# Autodesk Inventor assembly: 000-dribl-v2
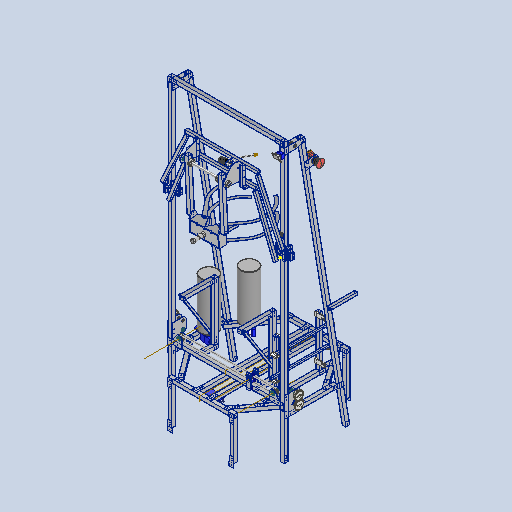
[picture p0: Inventor's stored thumbnail of the model, 512x512]
Saved by Autodesk Inventor 2025.2 (Build 292293000, 293)
## iProperties
Created: 2025-04-03
Part Number: 000-dribl-v2
Document SubType Name: Assembly
Designer: haruy
Author: haruy
## Documents named in this file (56)
- C:\Users\haruy\Documents\ロボコン\NHK2025\cad\nagahisa\dribl\000-dribl-v2.iam
- C:\Users\haruy\Documents\ロボコン\NHK2025\cad\nagahisa\dribl\dribl-v3-Sketch-Base.ipt
- C:\Users\haruy\Documents\ロボコン\NHK2025\cad\nagahisa\dribl\dribl-v1-Plate-5.ipt
- C:\Users\haruy\Documents\ロボコン\NHK2025\cad\nagahisa\dribl\dribl-v1-Plate-3.ipt
- C:\Users\haruy\Documents\ロボコン\NHK2025\cad\nagahisa\dribl\dribl-v1-Plate-4.ipt
- C:\Users\haruy\Documents\ロボコン\NHK2025\cad\nagahisa\dribl\dribl-v3-Plate-1.ipt
- C:\Users\haruy\Documents\ロボコン\NHK2025\cad\nagahisa\dribl\dribl-v3-Plate-2.ipt
- C:\Users\haruy\Documents\ロボコン\NHK2025\cad\nagahisa\dribl\dribl-v3-ASP-arm.ipt
- C:\Users\haruy\Documents\ロボコン\NHK2025\cad\nagahisa\dribl\dribl-v1-Shaft-spesa-57.ipt
- C:\Users\haruy\Documents\ロボコン\NHK2025\cad\nagahisa\dribl\dribl-v1-Plate-8.ipt
- C:\Users\haruy\Documents\ロボコン\NHK2025\cad\000_parts\モーター\robomaster\M2006 P36\RoboMaster M2006 P36\RoboMaster M2006 P36.ipt
- C:\Users\haruy\Documents\ロボコン\NHK2025\cad\nagahisa\dribl\dribl-v3-Plate-6.ipt
- C:\Users\haruy\Documents\ロボコン\NHK2025\cad\nagahisa\dribl\dribl-v3-Plate-7.ipt
- C:\Users\haruy\Documents\ロボコン\NHK2025\cad\nagahisa\dribl\dribl-v3-Plate-8.ipt
- C:\Users\haruy\Documents\ロボコン\NHK2025\cad\nagahisa\dribl\dribl-v3-Plate-9.ipt
- C:\Users\haruy\Documents\ロボコン\NHK2025\cad\nagahisa\dribl\dribl-v3-Plate-10.ipt
- C:\Users\haruy\Documents\ロボコン\NHK2025\cad\nagahisa\dribl\dribl-v3-Plate-11.ipt
- C:\Users\haruy\Documents\ロボコン\NHK2025\cad\nagahisa\dribl\dribl-v3-Plate-12.ipt
- C:\Users\haruy\Documents\ロボコン\NHK2025\cad\nagahisa\dribl\dribl-v3-ASP-1.ipt
- C:\Users\haruy\Documents\ロボコン\NHK2025\cad\nagahisa\dribl\dribl-v1-Plate-14.ipt
- C:\Users\haruy\Documents\ロボコン\NHK2025\cad\nagahisa\dribl\dribl-v1-3DP-P-F.ipt
- C:\Users\haruy\Documents\ロボコン\NHK2025\cad\nagahisa\dribl\roller-Base-v1-petbottle.ipt
- C:\Users\haruy\Documents\ロボコン\NHK2025\cad\nagahisa\dribl\dribl-v3-Plate-13.ipt
- C:\Users\haruy\Documents\ロボコン\NHK2025\cad\nagahisa\dribl\dribl-v3-Plate-14.ipt
- C:\Users\haruy\Documents\ロボコン\NHK2025\cad\nagahisa\base_weel\base_weel-v2-Plate-8.ipt
- C:\Users\haruy\Documents\ロボコン\NHK2025\cad\nagahisa\dribl\dribl-v3-ASP-2.ipt
- C:\Users\haruy\Documents\ロボコン\NHK2025\cad\nagahisa\base_weel\base_weel-v2-POM-pc-F-1.ipt
- C:\Users\haruy\Documents\ロボコン\NHK2025\cad\nagahisa\base_weel\base_weel-v2-POM-pc-F-2.ipt
- C:\Users\haruy\Documents\ロボコン\NHK2025\cad\nagahisa\dribl\dribl-v3-Plate-15.ipt
- C:\Users\haruy\Documents\ロボコン\NHK2025\cad\nagahisa\dribl\dribl-v1-Plate-13.ipt
- C:\Users\haruy\Documents\ロボコン\NHK2025\cad\000_parts\回路関連\EMO\emo_sa.ipt
- C:\Users\haruy\Documents\ロボコン\NHK2025\cad\nagahisa\dribl\dribl-v3-3DP-1.ipt
- C:\Users\haruy\Documents\ロボコン\NHK2025\cad\nagahisa\dribl\dribl-v3-Plate-16.ipt
- C:\Users\haruy\Documents\ロボコン\NHK2025\cad\nagahisa\dribl\000-dribl-v2\デザイン アクセラレータ\歯付きベルト伝達1.iam
- C:\Users\haruy\Documents\ロボコン\NHK2025\cad\000_parts\ベアリング\10\bear_10_15_sn.ipt
- C:\Users\haruy\Documents\ロボコン\NHK2025\cad\nagahisa\belt_liner\SCBRJ10-13.iam
- C:\Users\haruy\Documents\ロボコン\NHK2025\cad\nagahisa\dribl\dribl-v1-Plate-12.ipt
- C:\Users\haruy\Documents\ロボコン\NHK2025\cad\nagahisa\dribl\dribl-v1-3DP-l-F-1.ipt
- C:\Users\haruy\Documents\ロボコン\NHK2025\cad\000_parts\センサー\VX-012-1A3\VX-012-1A3\VX-012-1A3.iam
- C:\Users\haruy\Documents\ロボコン\NHK2025\cad\nagahisa\dribl\R2-Rzvector\TH22_bearing_12_18_19.5_sn.ipt
- C:\Users\haruy\Documents\ロボコン\NHK2025\cad\nagahisa\dribl\SCSNAJ12-16b.ipt
- C:\Users\haruy\Documents\ロボコン\NHK2025\cad\nagahisa\dribl\dribl-v1-Shaft-2.ipt
- C:\Users\haruy\Documents\ロボコン\NHK2025\cad\nagahisa\dribl\dribl-v3-3DP-2.ipt
- C:\Users\haruy\Documents\ロボコン\NHK2025\cad\000_parts\センサー\realsense\D435i_Solid.ipt
- C:\Users\haruy\Documents\ロボコン\NHK2025\cad\nagahisa\dribl\R2-Rzvector\bear_f8_12_sa.ipt
- C:\Users\haruy\Documents\ロボコン\NHK2025\cad\nagahisa\dribl\R2-Rzvector\bear_10_15_sn.ipt
- C:\Users\haruy\Documents\ロボコン\NHK2025\cad\nagahisa\dribl\SCTW12.iam
- C:\Users\haruy\Documents\ロボコン\NHK2025\cad\nagahisa\base_weel\SCSWA8-8.iam
- C:\Users\haruy\Documents\ロボコン\NHK2025\cad\nagahisa\belt_liner\SSCSW10-10b.ipt
- C:\Users\haruy\Documents\ロボコン\NHK2025\cad\nagahisa\dribl\000-dribl-v2\デザイン アクセラレータ\平歯車1.iam
- C:\Users\haruy\Documents\ロボコン\NHK2025\cad\nagahisa\dribl\000-dribl-v2\デザイン アクセラレータ\平歯車2.iam
- C:\Users\haruy\Documents\ロボコン\NHK2025\cad\nagahisa\hand\grab\hand-grab-v5-Plate-6.ipt
- C:\Users\haruy\Documents\ロボコン\NHK2025\cad\nagahisa\hand\grab\hand-grab-v5-Plate-7.ipt
- C:\Users\haruy\Documents\ロボコン\NHK2025\cad\nagahisa\hand\grab\000-hand-grab-v5.iam
- C:\Users\haruy\Documents\ロボコン\NHK2025\cad\nagahisa\hand\grab\hand-grab-v5-ASP-1.ipt
- C:\Users\haruy\Documents\ロボコン\NHK2025\cad\nagahisa\dribl\SCSW12-10.iam
## Components (113 placed, 53 different names)
1. dribl-v3-Sketch-Base:1 — 挿入:10, 挿入:11, 挿入:12, 挿入:13, 挿入:14, 挿入:15, 挿入:16, 挿入:17, 挿入:18, 挿入:19, 挿入:20, 挿入:21, 挿入:22, 挿入:23, 挿入:24, 挿入:25, 挿入:26, 挿入:27, 挿入:28, 挿入:29, 挿入:30, 挿入:31, 挿入:32, 挿入:33, 正接:1, 正接:2, 正接:3, 正接:4, 挿入:44, 挿入:45, 挿入:46, 挿入:47, 挿入:48, 挿入:49, 挿入:50, 挿入:51, 挿入:52, 挿入:53, 挿入:56, 挿入:57, 挿入:58, 挿入:59, 挿入:60, 挿入:61, 挿入:62, 挿入:63, 挿入:64, 挿入:65, 挿入:70, 挿入:71, 挿入:72, 挿入:73, 挿入:74, 挿入:75, 挿入:76, 挿入:77, 挿入:78, 挿入:79, 挿入:80, 挿入:81, 挿入:82, 挿入:83, 挿入:84, 挿入:85, 挿入:86, 挿入:87, 挿入:88, 挿入:89, 挿入:90, 挿入:91, 挿入:92, 挿入:93, 挿入:94, 挿入:95, 挿入:96, 挿入:97, メイト:3, メイト:4, メイト:5, メイト:6, 挿入:102, 挿入:103, 挿入:104, 挿入:105, 挿入:106, 挿入:107, 挿入:108, 挿入:109, 挿入:128, 挿入:129, 挿入:130, 挿入:131, 挿入:132, 挿入:133, 挿入:134, 挿入:135, 挿入:137, 挿入:138, 挿入:139, 挿入:140, フラッシュ:1, 挿入:149, 挿入:150, 挿入:151, 挿入:152, 挿入:163, 挿入:164
2. dribl-v1-Plate-5:1 — 挿入:12, 挿入:13, 挿入:173, 挿入:175
3. dribl-v1-Plate-5:2 — 挿入:10, 挿入:11, 挿入:174, 挿入:176
4. dribl-v1-Plate-3:1 — 挿入:14, 挿入:15, 挿入:167, 挿入:183
5. dribl-v1-Plate-4:1 — 挿入:16, 挿入:17, 挿入:168
6. dribl-v3-Plate-1:1 — 挿入:18, 挿入:19, 挿入:172
7. dribl-v3-Plate-1:2 — 挿入:20, 挿入:21, 挿入:171
8. dribl-v3-Plate-1:3 — 挿入:22, 挿入:23, 挿入:170
9. dribl-v3-Plate-1:4 — 挿入:24, 挿入:25, 挿入:169
10. dribl-v3-Plate-2:1 — 挿入:26, 挿入:27, 挿入:179
11. dribl-v3-Plate-2:2 — 挿入:28, 挿入:29, 挿入:180
12. dribl-v3-Plate-2:3 — 挿入:32, 挿入:33, 挿入:177
13. dribl-v3-Plate-2:4 — 挿入:30, 挿入:31, 挿入:178
14. dribl-v3-ASP-arm:1 — 正接:1, 正接:2, 正接:3, 正接:4, 挿入:202, 挿入:203, 挿入:204, 挿入:205
15. dribl-v1-Shaft-spesa-57:1 — 挿入:41, 挿入:206
16. dribl-v1-Shaft-spesa-57:2 — 挿入:208
17. dribl-v1-Shaft-spesa-57:3 — 挿入:42, 挿入:207
18. dribl-v1-Plate-8:1 — 挿入:41, 挿入:42, 挿入:43, 挿入:208
19. RoboMaster M2006 P36:1 — 挿入:43
20. dribl-v3-Plate-6:1 — 挿入:44, 挿入:45
21. dribl-v3-Plate-6:2 — 挿入:50, 挿入:51
22. dribl-v3-Plate-6:3 — 挿入:48, 挿入:49
23. dribl-v3-Plate-6:4 — 挿入:46, 挿入:47
24. dribl-v3-Plate-7:1 — 挿入:52, 挿入:53
25. dribl-v3-Plate-7:4 — 挿入:56, 挿入:57
26. dribl-v3-Plate-8:1 — 挿入:58, 挿入:59
27. dribl-v3-Plate-8:2 — 挿入:60, 挿入:61
28. dribl-v3-Plate-9:1 — 挿入:62, 挿入:63
29. dribl-v3-Plate-9:3 — 挿入:64, 挿入:65
30. dribl-v3-Plate-10:1 — 挿入:72, 挿入:73
31. dribl-v3-Plate-10:2 — 挿入:74, 挿入:75
32. dribl-v3-Plate-10:3 — 挿入:70, 挿入:71
33. dribl-v3-Plate-10:4 — 挿入:76, 挿入:77
34. dribl-v3-Plate-11:1 — 挿入:78, 挿入:79
35. dribl-v3-Plate-11:2 — 挿入:82, 挿入:83
36. dribl-v3-Plate-11:3 — 挿入:80, 挿入:81
37. dribl-v3-Plate-11:4 — 挿入:84, 挿入:85
38. dribl-v3-Plate-11:5 — 挿入:88, 挿入:89
39. dribl-v3-Plate-11:6 — 挿入:86, 挿入:87
40. dribl-v3-Plate-12:1 — 挿入:90, 挿入:91
41. dribl-v3-Plate-12:2 — 挿入:92, 挿入:93
42. dribl-v3-ASP-1:1 — 挿入:98, 挿入:99
43. dribl-v1-Plate-14:1 — 挿入:96, 挿入:97
44. dribl-v1-Plate-14:2 — 挿入:94, 挿入:95, 挿入:98, 挿入:99
45. dribl-v1-3DP-P-F:1 — 挿入:100, メイト:5, メイト:6
46. roller-Base-v1-petbottle:1 — 挿入:100
47. dribl-v1-3DP-P-F:2 — メイト:3, メイト:4, 挿入:101
48. roller-Base-v1-petbottle:2 — 挿入:101
49. dribl-v3-Plate-13:1 — 挿入:102, 挿入:103
50. dribl-v3-Plate-14:1 — 挿入:104, 挿入:105
51. base_weel-v2-Plate-8:1 — 挿入:106, 挿入:107, 挿入:110, 挿入:111
52. base_weel-v2-Plate-8:2 — 挿入:108, 挿入:109
53. dribl-v3-ASP-2:1 — 挿入:110, 挿入:111, 挿入:112, 挿入:113, 挿入:114, 挿入:115, 挿入:116, 挿入:117, 挿入:118, 挿入:119, 挿入:120, 挿入:121, 挿入:122, 挿入:123, 挿入:124, 挿入:125, 挿入:126, 挿入:127
54. base_weel-v2-POM-pc-F-1:1 — 挿入:112, 挿入:113
55. base_weel-v2-POM-pc-F-1:2 — 挿入:114, 挿入:115
56. base_weel-v2-POM-pc-F-2:1 — 挿入:118, 挿入:119
57. base_weel-v2-POM-pc-F-2:2 — 挿入:116, 挿入:117
58. base_weel-v2-POM-pc-F-2:3 — 挿入:122, 挿入:123
59. base_weel-v2-POM-pc-F-2:4 — 挿入:120, 挿入:121
60. base_weel-v2-POM-pc-F-1:3 — 挿入:126, 挿入:127
61. base_weel-v2-POM-pc-F-1:4 — 挿入:124, 挿入:125
62. dribl-v3-Plate-15:1 — 挿入:128, 挿入:129
63. dribl-v3-Plate-15:2 — 挿入:130, 挿入:131
64. dribl-v3-Plate-11:7 — 挿入:132, 挿入:133
65. dribl-v1-Plate-13:1 — 挿入:134, 挿入:135, 挿入:136
66. emo_sa:1 — 挿入:136
67. dribl-v3-3DP-1:1 — 挿入:139, 挿入:140, 挿入:143, 挿入:144
68. dribl-v3-3DP-1:2 — 挿入:137, 挿入:138, 挿入:141, 挿入:142
69. dribl-v3-Plate-16:1 — 挿入:143, 挿入:144
70. dribl-v3-Plate-16:2 — 挿入:141, 挿入:142
71. 歯付きベルト伝達:1 [sub-assembly] — 挿入:145, 挿入:146
72. bear_10_15_sn:1 — 挿入:145, 挿入:147
73. bear_10_15_sn:2 — 挿入:146, 挿入:148
74. SCBRJ10-13:1 [sub-assembly] — 挿入:147
75. SCBRJ10-13:2 [sub-assembly] — 挿入:148
76. dribl-v1-Plate-12:1 — 挿入:149, 挿入:150, 挿入:155, 挿入:156
77. dribl-v1-3DP-l-F-1:1 — 挿入:151, 挿入:152, 挿入:153, 挿入:154
78. VX-012-1A3:1 [sub-assembly] — 挿入:153, 挿入:154
79. VX-012-1A3:2 [sub-assembly] — 挿入:155, 挿入:156
80. TH22_bearing_12_18_19.5_sn:1 — 挿入:160, 挿入:210
81. TH22_bearing_12_18_19.5_sn:2 — 挿入:194, 挿入:209
82. SCSNAJ12-16b:1 — 挿入:194
83. SCSNAJ12-16b:2 — 挿入:160, 挿入:195
84. dribl-v1-Shaft-2:1 — 挿入:195
85. dribl-v3-3DP-2:1 — 挿入:163, 挿入:164, 挿入:165, 挿入:166
86. D435i_Solid:1 — 挿入:165, 挿入:166
87. TH22_bearing_12_18_19.5_sn:3 — 挿入:167, 挿入:184
88. TH22_bearing_12_18_19.5_sn:4 — 挿入:168
89. TH22_bearing_12_18_19.5_sn:5 — 挿入:170
90. TH22_bearing_12_18_19.5_sn:6 — 挿入:169
91. TH22_bearing_12_18_19.5_sn:7 — 挿入:171
92. TH22_bearing_12_18_19.5_sn:8 — 挿入:172
93. TH22_bearing_12_18_19.5_sn:9 — 挿入:173
94. TH22_bearing_12_18_19.5_sn:10 — 挿入:174, 挿入:181
95. bear_f8_12_sa:1 — 挿入:175
96. bear_f8_12_sa:2 — 挿入:176, 挿入:182
97. bear_10_15_sn:3 — 挿入:178
98. bear_10_15_sn:4 — 挿入:177
99. bear_10_15_sn:5 — 挿入:179
100. bear_10_15_sn:6 — 挿入:180
101. SCTW12:1 [sub-assembly] — 挿入:181, メイト:12
102. SCSWA8-8:1 [sub-assembly] — 挿入:182, メイト:10, メイト:11
103. SSCSW10-10b:1 — 挿入:183, メイト:9
104. SCTW12:2 [sub-assembly] — 挿入:184, メイト:7, メイト:8
105. 平歯車:1 [sub-assembly] — メイト:7, メイト:8, メイト:9
106. 平歯車:2 [sub-assembly] — メイト:10, メイト:11, メイト:12
107. hand-grab-v5-Plate-6:1 — 挿入:202, 挿入:203, 挿入:206, 挿入:207, 挿入:210, 挿入:211
108. hand-grab-v5-Plate-7:1 — 挿入:204, 挿入:205, 挿入:209
109. 000-hand-grab-v5:1 [sub-assembly] — 挿入:196, 挿入:197, 挿入:198, 挿入:199
110. hand-grab-v5-ASP-1:1 — 挿入:196, 挿入:197, 挿入:200
111. hand-grab-v5-ASP-1:2 — 挿入:198, 挿入:199, 挿入:201, 挿入:211
112. SCSW12-10:1 [sub-assembly] — 挿入:201
113. SCSW12-10:2 [sub-assembly] — 挿入:200
## Relationships (190: Insert 175, Mate 10, Tangent 4, Flush 1)
- 挿入:10 [Insert]: dribl-v3-Sketch-Base:1 ↔ dribl-v1-Plate-5:2
- 挿入:11 [Insert]: dribl-v3-Sketch-Base:1 ↔ dribl-v1-Plate-5:2
- 挿入:12 [Insert]: dribl-v3-Sketch-Base:1 ↔ dribl-v1-Plate-5:1
- 挿入:13 [Insert]: dribl-v3-Sketch-Base:1 ↔ dribl-v1-Plate-5:1
- 挿入:14 [Insert]: dribl-v3-Sketch-Base:1 ↔ dribl-v1-Plate-3:1
- 挿入:15 [Insert]: dribl-v3-Sketch-Base:1 ↔ dribl-v1-Plate-3:1
- 挿入:16 [Insert]: dribl-v3-Sketch-Base:1 ↔ dribl-v1-Plate-4:1
- 挿入:17 [Insert]: dribl-v3-Sketch-Base:1 ↔ dribl-v1-Plate-4:1
- 挿入:18 [Insert]: dribl-v3-Sketch-Base:1 ↔ dribl-v3-Plate-1:1
- 挿入:19 [Insert]: dribl-v3-Sketch-Base:1 ↔ dribl-v3-Plate-1:1
- 挿入:20 [Insert]: dribl-v3-Sketch-Base:1 ↔ dribl-v3-Plate-1:2
- 挿入:21 [Insert]: dribl-v3-Sketch-Base:1 ↔ dribl-v3-Plate-1:2
- 挿入:22 [Insert]: dribl-v3-Sketch-Base:1 ↔ dribl-v3-Plate-1:3
- 挿入:23 [Insert]: dribl-v3-Sketch-Base:1 ↔ dribl-v3-Plate-1:3
- 挿入:24 [Insert]: dribl-v3-Sketch-Base:1 ↔ dribl-v3-Plate-1:4
- 挿入:25 [Insert]: dribl-v3-Sketch-Base:1 ↔ dribl-v3-Plate-1:4
- 挿入:26 [Insert]: dribl-v3-Sketch-Base:1 ↔ dribl-v3-Plate-2:1
- 挿入:27 [Insert]: dribl-v3-Sketch-Base:1 ↔ dribl-v3-Plate-2:1
- 挿入:28 [Insert]: dribl-v3-Sketch-Base:1 ↔ dribl-v3-Plate-2:2
- 挿入:29 [Insert]: dribl-v3-Sketch-Base:1 ↔ dribl-v3-Plate-2:2
- 挿入:30 [Insert]: dribl-v3-Sketch-Base:1 ↔ dribl-v3-Plate-2:4
- 挿入:31 [Insert]: dribl-v3-Sketch-Base:1 ↔ dribl-v3-Plate-2:4
- 挿入:32 [Insert]: dribl-v3-Sketch-Base:1 ↔ dribl-v3-Plate-2:3
- 挿入:33 [Insert]: dribl-v3-Sketch-Base:1 ↔ dribl-v3-Plate-2:3
- 正接:1 [Tangent]: dribl-v3-Sketch-Base:1 ↔ dribl-v3-ASP-arm:1
- 正接:2 [Tangent]: dribl-v3-Sketch-Base:1 ↔ dribl-v3-ASP-arm:1
- 正接:3 [Tangent]: dribl-v3-Sketch-Base:1 ↔ dribl-v3-ASP-arm:1
- 正接:4 [Tangent]: dribl-v3-Sketch-Base:1 ↔ dribl-v3-ASP-arm:1
- 挿入:41 [Insert]: dribl-v1-Shaft-spesa-57:1 ↔ dribl-v1-Plate-8:1
- 挿入:42 [Insert]: dribl-v1-Shaft-spesa-57:3 ↔ dribl-v1-Plate-8:1
- 挿入:43 [Insert]: dribl-v1-Plate-8:1 ↔ RoboMaster M2006 P36:1
- 挿入:44 [Insert]: dribl-v3-Sketch-Base:1 ↔ dribl-v3-Plate-6:1
- 挿入:45 [Insert]: dribl-v3-Sketch-Base:1 ↔ dribl-v3-Plate-6:1
- 挿入:46 [Insert]: dribl-v3-Sketch-Base:1 ↔ dribl-v3-Plate-6:4
- 挿入:47 [Insert]: dribl-v3-Sketch-Base:1 ↔ dribl-v3-Plate-6:4
- 挿入:48 [Insert]: dribl-v3-Sketch-Base:1 ↔ dribl-v3-Plate-6:3
- 挿入:49 [Insert]: dribl-v3-Sketch-Base:1 ↔ dribl-v3-Plate-6:3
- 挿入:50 [Insert]: dribl-v3-Sketch-Base:1 ↔ dribl-v3-Plate-6:2
- 挿入:51 [Insert]: dribl-v3-Sketch-Base:1 ↔ dribl-v3-Plate-6:2
- 挿入:52 [Insert]: dribl-v3-Sketch-Base:1 ↔ dribl-v3-Plate-7:1
- 挿入:53 [Insert]: dribl-v3-Sketch-Base:1 ↔ dribl-v3-Plate-7:1
- 挿入:56 [Insert]: dribl-v3-Sketch-Base:1 ↔ dribl-v3-Plate-7:4
- 挿入:57 [Insert]: dribl-v3-Sketch-Base:1 ↔ dribl-v3-Plate-7:4
- 挿入:58 [Insert]: dribl-v3-Sketch-Base:1 ↔ dribl-v3-Plate-8:1
- 挿入:59 [Insert]: dribl-v3-Sketch-Base:1 ↔ dribl-v3-Plate-8:1
- 挿入:60 [Insert]: dribl-v3-Sketch-Base:1 ↔ dribl-v3-Plate-8:2
- 挿入:61 [Insert]: dribl-v3-Sketch-Base:1 ↔ dribl-v3-Plate-8:2
- 挿入:62 [Insert]: dribl-v3-Sketch-Base:1 ↔ dribl-v3-Plate-9:1
- 挿入:63 [Insert]: dribl-v3-Sketch-Base:1 ↔ dribl-v3-Plate-9:1
- 挿入:64 [Insert]: dribl-v3-Sketch-Base:1 ↔ dribl-v3-Plate-9:3
- 挿入:65 [Insert]: dribl-v3-Sketch-Base:1 ↔ dribl-v3-Plate-9:3
- 挿入:70 [Insert]: dribl-v3-Sketch-Base:1 ↔ dribl-v3-Plate-10:3
- 挿入:71 [Insert]: dribl-v3-Sketch-Base:1 ↔ dribl-v3-Plate-10:3
- 挿入:72 [Insert]: dribl-v3-Sketch-Base:1 ↔ dribl-v3-Plate-10:1
- 挿入:73 [Insert]: dribl-v3-Sketch-Base:1 ↔ dribl-v3-Plate-10:1
- 挿入:74 [Insert]: dribl-v3-Sketch-Base:1 ↔ dribl-v3-Plate-10:2
- 挿入:75 [Insert]: dribl-v3-Sketch-Base:1 ↔ dribl-v3-Plate-10:2
- 挿入:76 [Insert]: dribl-v3-Sketch-Base:1 ↔ dribl-v3-Plate-10:4
- 挿入:77 [Insert]: dribl-v3-Sketch-Base:1 ↔ dribl-v3-Plate-10:4
- 挿入:78 [Insert]: dribl-v3-Sketch-Base:1 ↔ dribl-v3-Plate-11:1
- 挿入:79 [Insert]: dribl-v3-Sketch-Base:1 ↔ dribl-v3-Plate-11:1
- 挿入:80 [Insert]: dribl-v3-Sketch-Base:1 ↔ dribl-v3-Plate-11:3
- 挿入:81 [Insert]: dribl-v3-Sketch-Base:1 ↔ dribl-v3-Plate-11:3
- 挿入:82 [Insert]: dribl-v3-Sketch-Base:1 ↔ dribl-v3-Plate-11:2
- 挿入:83 [Insert]: dribl-v3-Sketch-Base:1 ↔ dribl-v3-Plate-11:2
- 挿入:84 [Insert]: dribl-v3-Sketch-Base:1 ↔ dribl-v3-Plate-11:4
- 挿入:85 [Insert]: dribl-v3-Sketch-Base:1 ↔ dribl-v3-Plate-11:4
- 挿入:86 [Insert]: dribl-v3-Sketch-Base:1 ↔ dribl-v3-Plate-11:6
- 挿入:87 [Insert]: dribl-v3-Sketch-Base:1 ↔ dribl-v3-Plate-11:6
- 挿入:88 [Insert]: dribl-v3-Sketch-Base:1 ↔ dribl-v3-Plate-11:5
- 挿入:89 [Insert]: dribl-v3-Sketch-Base:1 ↔ dribl-v3-Plate-11:5
- 挿入:90 [Insert]: dribl-v3-Sketch-Base:1 ↔ dribl-v3-Plate-12:1
- 挿入:91 [Insert]: dribl-v3-Sketch-Base:1 ↔ dribl-v3-Plate-12:1
- 挿入:92 [Insert]: dribl-v3-Sketch-Base:1 ↔ dribl-v3-Plate-12:2
- 挿入:93 [Insert]: dribl-v3-Sketch-Base:1 ↔ dribl-v3-Plate-12:2
- 挿入:94 [Insert]: dribl-v3-Sketch-Base:1 ↔ dribl-v1-Plate-14:2
- 挿入:95 [Insert]: dribl-v3-Sketch-Base:1 ↔ dribl-v1-Plate-14:2
- 挿入:96 [Insert]: dribl-v3-Sketch-Base:1 ↔ dribl-v1-Plate-14:1
- 挿入:97 [Insert]: dribl-v3-Sketch-Base:1 ↔ dribl-v1-Plate-14:1
- 挿入:98 [Insert]: dribl-v3-ASP-1:1 ↔ dribl-v1-Plate-14:2
- 挿入:99 [Insert]: dribl-v3-ASP-1:1 ↔ dribl-v1-Plate-14:2
- 挿入:100 [Insert]: dribl-v1-3DP-P-F:1 ↔ roller-Base-v1-petbottle:1
- メイト:3 [Mate]: dribl-v3-Sketch-Base:1 ↔ dribl-v1-3DP-P-F:2
- メイト:4 [Mate]: dribl-v3-Sketch-Base:1 ↔ dribl-v1-3DP-P-F:2
- 挿入:101 [Insert]: dribl-v1-3DP-P-F:2 ↔ roller-Base-v1-petbottle:2
- メイト:5 [Mate]: dribl-v3-Sketch-Base:1 ↔ dribl-v1-3DP-P-F:1
- メイト:6 [Mate]: dribl-v3-Sketch-Base:1 ↔ dribl-v1-3DP-P-F:1
- 挿入:102 [Insert]: dribl-v3-Sketch-Base:1 ↔ dribl-v3-Plate-13:1
- 挿入:103 [Insert]: dribl-v3-Sketch-Base:1 ↔ dribl-v3-Plate-13:1
- 挿入:104 [Insert]: dribl-v3-Sketch-Base:1 ↔ dribl-v3-Plate-14:1
- 挿入:105 [Insert]: dribl-v3-Sketch-Base:1 ↔ dribl-v3-Plate-14:1
- 挿入:106 [Insert]: dribl-v3-Sketch-Base:1 ↔ base_weel-v2-Plate-8:1
- 挿入:107 [Insert]: dribl-v3-Sketch-Base:1 ↔ base_weel-v2-Plate-8:1
- 挿入:108 [Insert]: dribl-v3-Sketch-Base:1 ↔ base_weel-v2-Plate-8:2
- 挿入:109 [Insert]: dribl-v3-Sketch-Base:1 ↔ base_weel-v2-Plate-8:2
- 挿入:110 [Insert]: base_weel-v2-Plate-8:1 ↔ dribl-v3-ASP-2:1
- 挿入:111 [Insert]: base_weel-v2-Plate-8:1 ↔ dribl-v3-ASP-2:1
- 挿入:112 [Insert]: dribl-v3-ASP-2:1 ↔ base_weel-v2-POM-pc-F-1:1
- 挿入:113 [Insert]: dribl-v3-ASP-2:1 ↔ base_weel-v2-POM-pc-F-1:1
- 挿入:114 [Insert]: dribl-v3-ASP-2:1 ↔ base_weel-v2-POM-pc-F-1:2
- 挿入:115 [Insert]: dribl-v3-ASP-2:1 ↔ base_weel-v2-POM-pc-F-1:2
- 挿入:116 [Insert]: dribl-v3-ASP-2:1 ↔ base_weel-v2-POM-pc-F-2:2
- 挿入:117 [Insert]: dribl-v3-ASP-2:1 ↔ base_weel-v2-POM-pc-F-2:2
- 挿入:118 [Insert]: dribl-v3-ASP-2:1 ↔ base_weel-v2-POM-pc-F-2:1
- 挿入:119 [Insert]: dribl-v3-ASP-2:1 ↔ base_weel-v2-POM-pc-F-2:1
- 挿入:120 [Insert]: dribl-v3-ASP-2:1 ↔ base_weel-v2-POM-pc-F-2:4
- 挿入:121 [Insert]: dribl-v3-ASP-2:1 ↔ base_weel-v2-POM-pc-F-2:4
- 挿入:122 [Insert]: dribl-v3-ASP-2:1 ↔ base_weel-v2-POM-pc-F-2:3
- 挿入:123 [Insert]: dribl-v3-ASP-2:1 ↔ base_weel-v2-POM-pc-F-2:3
- 挿入:124 [Insert]: dribl-v3-ASP-2:1 ↔ base_weel-v2-POM-pc-F-1:4
- 挿入:125 [Insert]: dribl-v3-ASP-2:1 ↔ base_weel-v2-POM-pc-F-1:4
- 挿入:126 [Insert]: dribl-v3-ASP-2:1 ↔ base_weel-v2-POM-pc-F-1:3
- 挿入:127 [Insert]: dribl-v3-ASP-2:1 ↔ base_weel-v2-POM-pc-F-1:3
- 挿入:128 [Insert]: dribl-v3-Sketch-Base:1 ↔ dribl-v3-Plate-15:1
- 挿入:129 [Insert]: dribl-v3-Sketch-Base:1 ↔ dribl-v3-Plate-15:1
- 挿入:130 [Insert]: dribl-v3-Sketch-Base:1 ↔ dribl-v3-Plate-15:2
- 挿入:131 [Insert]: dribl-v3-Sketch-Base:1 ↔ dribl-v3-Plate-15:2
- 挿入:132 [Insert]: dribl-v3-Sketch-Base:1 ↔ dribl-v3-Plate-11:7
- 挿入:133 [Insert]: dribl-v3-Sketch-Base:1 ↔ dribl-v3-Plate-11:7
- 挿入:134 [Insert]: dribl-v3-Sketch-Base:1 ↔ dribl-v1-Plate-13:1
- 挿入:135 [Insert]: dribl-v3-Sketch-Base:1 ↔ dribl-v1-Plate-13:1
- 挿入:136 [Insert]: dribl-v1-Plate-13:1 ↔ emo_sa:1
- 挿入:137 [Insert]: dribl-v3-Sketch-Base:1 ↔ dribl-v3-3DP-1:2
- 挿入:138 [Insert]: dribl-v3-Sketch-Base:1 ↔ dribl-v3-3DP-1:2
- 挿入:139 [Insert]: dribl-v3-Sketch-Base:1 ↔ dribl-v3-3DP-1:1
- 挿入:140 [Insert]: dribl-v3-Sketch-Base:1 ↔ dribl-v3-3DP-1:1
- 挿入:141 [Insert]: dribl-v3-3DP-1:2 ↔ dribl-v3-Plate-16:2
- 挿入:142 [Insert]: dribl-v3-3DP-1:2 ↔ dribl-v3-Plate-16:2
- 挿入:143 [Insert]: dribl-v3-3DP-1:1 ↔ dribl-v3-Plate-16:1
- 挿入:144 [Insert]: dribl-v3-3DP-1:1 ↔ dribl-v3-Plate-16:1
- フラッシュ:1 [Flush] (-10 mm): dribl-v3-Sketch-Base:1
- 挿入:145 [Insert]: 歯付きベルト伝達:1 ↔ bear_10_15_sn:1
- 挿入:146 [Insert]: 歯付きベルト伝達:1 ↔ bear_10_15_sn:2
- 挿入:147 [Insert]: bear_10_15_sn:1 ↔ SCBRJ10-13:1
- 挿入:148 [Insert]: bear_10_15_sn:2 ↔ SCBRJ10-13:2
- 挿入:149 [Insert]: dribl-v3-Sketch-Base:1 ↔ dribl-v1-Plate-12:1
- 挿入:150 [Insert]: dribl-v3-Sketch-Base:1 ↔ dribl-v1-Plate-12:1
- 挿入:151 [Insert]: dribl-v3-Sketch-Base:1 ↔ dribl-v1-3DP-l-F-1:1
- 挿入:152 [Insert]: dribl-v3-Sketch-Base:1 ↔ dribl-v1-3DP-l-F-1:1
- 挿入:153 [Insert]: dribl-v1-3DP-l-F-1:1 ↔ VX-012-1A3:1
- 挿入:154 [Insert]: dribl-v1-3DP-l-F-1:1 ↔ VX-012-1A3:1
- 挿入:155 [Insert]: dribl-v1-Plate-12:1 ↔ VX-012-1A3:2
- 挿入:156 [Insert]: dribl-v1-Plate-12:1 ↔ VX-012-1A3:2
- 挿入:160 [Insert]: TH22_bearing_12_18_19.5_sn:1 ↔ SCSNAJ12-16b:2
- 挿入:163 [Insert]: dribl-v3-Sketch-Base:1 ↔ dribl-v3-3DP-2:1
- 挿入:164 [Insert]: dribl-v3-Sketch-Base:1 ↔ dribl-v3-3DP-2:1
- 挿入:165 [Insert]: dribl-v3-3DP-2:1 ↔ D435i_Solid:1
- 挿入:166 [Insert]: dribl-v3-3DP-2:1 ↔ D435i_Solid:1
- 挿入:167 [Insert]: dribl-v1-Plate-3:1 ↔ TH22_bearing_12_18_19.5_sn:3
- 挿入:168 [Insert]: dribl-v1-Plate-4:1 ↔ TH22_bearing_12_18_19.5_sn:4
- 挿入:169 [Insert]: dribl-v3-Plate-1:4 ↔ TH22_bearing_12_18_19.5_sn:6
- 挿入:170 [Insert]: dribl-v3-Plate-1:3 ↔ TH22_bearing_12_18_19.5_sn:5
- 挿入:171 [Insert]: dribl-v3-Plate-1:2 ↔ TH22_bearing_12_18_19.5_sn:7
- 挿入:172 [Insert]: dribl-v3-Plate-1:1 ↔ TH22_bearing_12_18_19.5_sn:8
- 挿入:173 [Insert]: dribl-v1-Plate-5:1 ↔ TH22_bearing_12_18_19.5_sn:9
- 挿入:174 [Insert]: dribl-v1-Plate-5:2 ↔ TH22_bearing_12_18_19.5_sn:10
- 挿入:175 [Insert]: dribl-v1-Plate-5:1 ↔ bear_f8_12_sa:1
- 挿入:176 [Insert]: dribl-v1-Plate-5:2 ↔ bear_f8_12_sa:2
- 挿入:177 [Insert]: dribl-v3-Plate-2:3 ↔ bear_10_15_sn:4
- 挿入:178 [Insert]: dribl-v3-Plate-2:4 ↔ bear_10_15_sn:3
- 挿入:179 [Insert]: dribl-v3-Plate-2:1 ↔ bear_10_15_sn:5
- 挿入:180 [Insert]: dribl-v3-Plate-2:2 ↔ bear_10_15_sn:6
- 挿入:181 [Insert] (5 mm): TH22_bearing_12_18_19.5_sn:10 ↔ SCTW12:1
- 挿入:182 [Insert] (9.3 mm): bear_f8_12_sa:2 ↔ SCSWA8-8:1
- 挿入:183 [Insert] (7 mm): dribl-v1-Plate-3:1 ↔ SSCSW10-10b:1
- 挿入:184 [Insert] (4 mm): TH22_bearing_12_18_19.5_sn:3 ↔ SCTW12:2
- メイト:7 [Mate]: SCTW12:2 ↔ 平歯車:1
- メイト:8 [Mate]: SCTW12:2 ↔ 平歯車:1
- メイト:9 [Mate]: SSCSW10-10b:1 ↔ 平歯車:1
- メイト:10 [Mate]: SCSWA8-8:1 ↔ 平歯車:2
- メイト:11 [Mate]: SCSWA8-8:1 ↔ 平歯車:2
- メイト:12 [Mate]: SCTW12:1 ↔ 平歯車:2
- 挿入:194 [Insert]: TH22_bearing_12_18_19.5_sn:2 ↔ SCSNAJ12-16b:1
- 挿入:195 [Insert]: SCSNAJ12-16b:2 ↔ dribl-v1-Shaft-2:1
- 挿入:196 [Insert]: 000-hand-grab-v5:1 ↔ hand-grab-v5-ASP-1:1
- 挿入:197 [Insert]: 000-hand-grab-v5:1 ↔ hand-grab-v5-ASP-1:1
- 挿入:198 [Insert]: 000-hand-grab-v5:1 ↔ hand-grab-v5-ASP-1:2
- 挿入:199 [Insert]: 000-hand-grab-v5:1 ↔ hand-grab-v5-ASP-1:2
- 挿入:200 [Insert]: hand-grab-v5-ASP-1:1 ↔ SCSW12-10:2
- 挿入:201 [Insert]: hand-grab-v5-ASP-1:2 ↔ SCSW12-10:1
- 挿入:202 [Insert]: dribl-v3-ASP-arm:1 ↔ hand-grab-v5-Plate-6:1
- 挿入:203 [Insert]: dribl-v3-ASP-arm:1 ↔ hand-grab-v5-Plate-6:1
- 挿入:204 [Insert]: dribl-v3-ASP-arm:1 ↔ hand-grab-v5-Plate-7:1
- 挿入:205 [Insert]: dribl-v3-ASP-arm:1 ↔ hand-grab-v5-Plate-7:1
- 挿入:206 [Insert]: dribl-v1-Shaft-spesa-57:1 ↔ hand-grab-v5-Plate-6:1
- 挿入:207 [Insert]: dribl-v1-Shaft-spesa-57:3 ↔ hand-grab-v5-Plate-6:1
- 挿入:208 [Insert]: dribl-v1-Shaft-spesa-57:2 ↔ dribl-v1-Plate-8:1
- 挿入:209 [Insert]: TH22_bearing_12_18_19.5_sn:2 ↔ hand-grab-v5-Plate-7:1
- 挿入:210 [Insert]: TH22_bearing_12_18_19.5_sn:1 ↔ hand-grab-v5-Plate-6:1
- 挿入:211 [Insert] (13 mm): hand-grab-v5-Plate-6:1 ↔ hand-grab-v5-ASP-1:2
